# Autodesk Inventor assembly: foiurbar
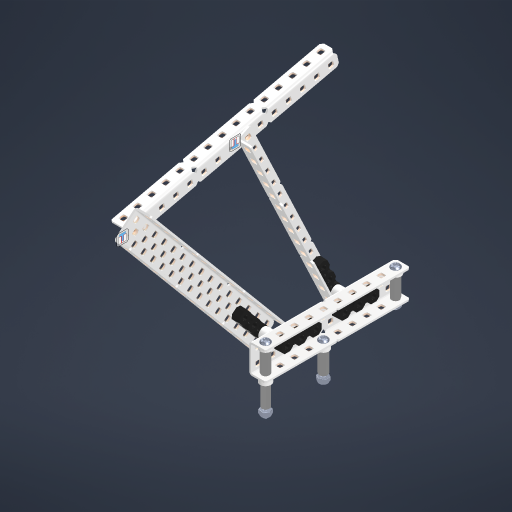
[picture p0: Inventor's stored thumbnail of the model, 512x512]
Saved by Autodesk Inventor 2023 (Build 270158000, 158)
## iProperties
Created: 2023-08-08
Part Number: foiurbar
Document SubType Name: Assembly
Designer: srbel
Author: srbel
## Documents named in this file (15)
- C:\CAD\OverUnderCAD\Drive\foiurbar.iam
- C:\CAD\OverUnderCAD\VEX-CAD-Inventor-1.4.0\Structure\C Channel\Aluminum 1x2x1\Alu C 1x2x1x10.ipt
- C:\CAD\OverUnderCAD\VEX-CAD-Inventor-1.4.0\Motion\Spacers\Spacer Nylon .313 OD\NSpacer .313 OD x .125.ipt
- C:\CAD\OverUnderCAD\VEX-CAD-Inventor-1.4.0\Motion\Spacers\Spacer Nylon .313 OD.ipt
- C:\CAD\OverUnderCAD\VEX-CAD-Inventor-1.4.0\Structure\Standoff\Standoff .75.ipt
- C:\CAD\OverUnderCAD\VEX-CAD-Inventor-1.4.0\Structure\Standoff.ipt
- C:\CAD\OverUnderCAD\VEX-CAD-Inventor-1.4.0\Structure\Hardware\Screw Steel - Star\SScrew Star Threaded 2.250.ipt
- C:\CAD\OverUnderCAD\VEX-CAD-Inventor-1.4.0\Structure\Hardware\Screw Steel - Star.ipt
- C:\CAD\OverUnderCAD\VEX-CAD-Inventor-1.4.0\Structure\Hardware\Nut Thin Nylock.ipt
- C:\CAD\OverUnderCAD\VEX-CAD-Inventor-1.4.0\Structure\Hardware\Screw Steel - Star\SScrew Star Threaded 1.250.ipt
- C:\CAD\OverUnderCAD\VEX-CAD-Inventor-1.4.0\Motion\Shaft LS\Bearing Flat.ipt
- C:\CAD\OverUnderCAD\VEX-CAD-Inventor-1.4.0\Structure\C Channel\Aluminum 1x2x1\Alu C 1x2x1x15.ipt
- C:\CAD\OverUnderCAD\VEX-CAD-Inventor-1.4.0\Motion\Spacers\Spacer Nylon .313 OD\NSpacer .313 OD x .500.ipt
- C:\CAD\OverUnderCAD\VEX-CAD-Inventor-1.4.0\Structure\Angle\Aluminum\1x1\Alu Angle 1x1x14.ipt
- C:\CAD\OverUnderCAD\VEX-CAD-Inventor-1.4.0\Structure\Angle\Aluminum\1x1\Alu Angle 1x1x15.ipt
## Components (24 placed, 11 different names)
1. Alu C 1x2x1x10:1 — Insert:16, Insert:17, Insert:18, Insert:19, Insert:20, Insert:49, Insert:50
2. NSpacer .313 OD x .125:1
3. Standoff .75:1
4. NSpacer .313 OD x .125:2
5. Standoff .75:2
6. Standoff .75:3 — Insert:15
7. NSpacer .313 OD x .125:3
8. Standoff .75:4
9. SScrew Star Threaded 2.250:1
10. Nut Thin Nylock:1
11. Nut Thin Nylock:2
12. Nut Thin Nylock:3
13. SScrew Star Threaded 1.250:2
14. NSpacer .313 OD x .125:5 — Insert:15, Insert:16
15. Bearing Flat:1 — Insert:17, Insert:18
16. Bearing Flat:2 — Insert:19
17. SScrew Star Threaded 1.250:3 — Insert:20
18. Alu Angle 1x1x14:1 — Insert:46, Insert:47, Insert:52
19. Alu C 1x2x1x15:1 — Insert:43, Insert:44, Insert:51
20. Bearing Flat:5 — Insert:43, Insert:44, Insert:45
21. NSpacer .313 OD x .500:12 — Insert:45, Insert:50
22. Bearing Flat:6 — Insert:46, Insert:47, Insert:48
23. NSpacer .313 OD x .500:16 — Insert:48, Insert:49
24. Alu Angle 1x1x15:1 — Insert:51, Insert:52
## Relationships (27: Insert 27)
- [Insert]: NSpacer .313 OD x .125:1 ↔ Standoff .75:1
- [Insert]: Alu C 1x2x1x10:1 ↔ NSpacer .313 OD x .125:1
- [Insert]: NSpacer .313 OD x .125:2 ↔ Standoff .75:2
- [Insert]: Alu C 1x2x1x10:1 ↔ NSpacer .313 OD x .125:2
- [Insert]: NSpacer .313 OD x .125:3 ↔ Standoff .75:4
- [Insert] (1.5875 mm): Alu C 1x2x1x10:1 ↔ NSpacer .313 OD x .125:3
- [Insert]: Alu C 1x2x1x10:1 ↔ SScrew Star Threaded 2.250:1
- [Insert] (1.5875 mm): Standoff .75:3 ↔ Nut Thin Nylock:2
- [Insert] (1.5875 mm): Standoff .75:4 ↔ Nut Thin Nylock:1
- [Insert]: Alu C 1x2x1x10:1 ↔ Nut Thin Nylock:3
- [Insert]: Alu C 1x2x1x10:1 ↔ SScrew Star Threaded 1.250:2
- Insert:15: Standoff .75:3 ↔ NSpacer .313 OD x .125:5
- Insert:16 (1.5875 mm): Alu C 1x2x1x10:1 ↔ NSpacer .313 OD x .125:5
- Insert:17: Alu C 1x2x1x10:1 ↔ Bearing Flat:1
- Insert:18: Alu C 1x2x1x10:1 ↔ Bearing Flat:1
- Insert:19: Alu C 1x2x1x10:1 ↔ Bearing Flat:2
- Insert:20: Alu C 1x2x1x10:1 ↔ SScrew Star Threaded 1.250:3
- Insert:43: Alu C 1x2x1x15:1 ↔ Bearing Flat:5
- Insert:44: Alu C 1x2x1x15:1 ↔ Bearing Flat:5
- Insert:45: Bearing Flat:5 ↔ NSpacer .313 OD x .500:12
- Insert:46: Alu Angle 1x1x14:1 ↔ Bearing Flat:6
- Insert:47: Alu Angle 1x1x14:1 ↔ Bearing Flat:6
- Insert:48: Bearing Flat:6 ↔ NSpacer .313 OD x .500:16
- Insert:49: Alu C 1x2x1x10:1 ↔ NSpacer .313 OD x .500:16
- Insert:50: Alu C 1x2x1x10:1 ↔ NSpacer .313 OD x .500:12
- Insert:51: Alu C 1x2x1x15:1 ↔ Alu Angle 1x1x15:1
- Insert:52: Alu Angle 1x1x14:1 ↔ Alu Angle 1x1x15:1
## Named parameters: d288_d1 = 0 mm, d290_d1 = 0 mm, d294_d292_d1 = 0 mm
